# Autodesk Inventor assembly: LeftArm
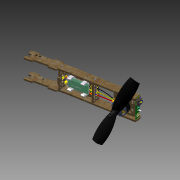
[picture p0: Inventor's stored thumbnail of the model, 180x180]
Saved by Autodesk Inventor 2012 (Build 160160000, 160)
## iProperties
Created: 2014-07-20
Part Number: LeftArm
Document SubType Name: Assembly
Designer: Anon
Author: Anon
## Documents named in this file (12)
- D:\Dropbox\Courses\GP\Inventor\dronestructure\LeftArm.iam
- D:\Dropbox\Courses\GP\Inventor\dronestructure\MotorCableHolder.ipt
- D:\Dropbox\Courses\GP\Inventor\dronestructure\ESCcableHolder.ipt
- D:\Dropbox\Courses\GP\Inventor\dronestructure\ArmOutside.ipt
- D:\Dropbox\Courses\GP\Inventor\dronestructure\ArmInsideLow.ipt
- C:\Users\Anon\Documents\Inventor\Content Center Files\R2012\en-US\ISO 4032(2)\ISO 4032 - M2,5ISO.ipt
- C:\Users\Anon\Documents\Inventor\Content Center Files\R2012\en-US\ISO 1207(1)\ISO 1207 - M2,5 x 14DIN EN ISO.ipt
- D:\Dropbox\Courses\GP\Inventor\dronestructure\electronics\afroesc\escassembly.iam
- D:\Dropbox\Courses\GP\Inventor\dronestructure\motor\motormounted.iam
- D:\Dropbox\Courses\GP\Inventor\dronestructure\LeftArm\AIP\Cable and Harness\LeftArm.MotorCables.iam
- D:\Dropbox\Courses\GP\Inventor\dronestructure\electronics\wingleds\wingledpcb\WingLeds.iam
- D:\Dropbox\Courses\GP\Inventor\dronestructure\CrimpSocket.ipt
## Components (21 placed, 11 different names)
1. MotorCableHolder:1 — Mate:19, Mate:21, Mate:27, Flush:3, Mate:28
2. ESCcableHolder:1 — Flush:1, Mate:1, Mate:2, Mate:4, Mate:5, Flush:2, Mate:11, Mate:23, Flush:5, Flush:6, Flush:7
3. ArmOutside:1 — Flush:1, Mate:1, Mate:2, Mate:8, Mate:9, Mate:12, Mate:13, Mate:25, Mate:26, Flush:3, Mate:28, Mate:31, Mate:34, Mate:35, Mate:41, Flush:4
4. ArmInsideLow:1 — Mate:4, Mate:5, Flush:2, Mate:14, Mate:15, Mate:16, Mate:17, Mate:24, Mate:27, Mate:29, Mate:30, Mate:32, Mate:33, Mate:40
5. ISO 4032 M2,5:1 — Mate:10, Mate:11
6. ISO 4032 M2,5:2 — Mate:18, Mate:19
7. ISO 4032 M2,5:3 — Mate:22, Mate:23
8. ISO 4032 M2,5:4 — Mate:20, Mate:21
9. DIN EN ISO 1207 M2,5 x 14:1 — Mate:8, Mate:9, Mate:10
10. DIN EN ISO 1207 M2,5 x 14:2 — Mate:12, Mate:13, Mate:18
11. DIN EN ISO 1207 M2,5 x 14:3 — Mate:14, Mate:15, Mate:22
12. DIN EN ISO 1207 M2,5 x 14:4 — Mate:16, Mate:17, Mate:20
13. ESC [sub-assembly] — Mate:24, Mate:25, Mate:26
14. Motor [sub-assembly] — Mate:29, Mate:30, Mate:31, Mate:37, Mate:39
15. LeftArm.MotorCables [sub-assembly]
16. DIN EN ISO 1207 M2,5 x 14:5 — Mate:32, Mate:33, Mate:38
17. DIN EN ISO 1207 M2,5 x 14:6 — Mate:34, Mate:35, Mate:36
18. ISO 4032 M2,5:5 — Mate:36, Mate:37
19. ISO 4032 M2,5:6 — Mate:38, Mate:39
20. WingLEDs [sub-assembly] — Mate:40, Mate:41, Flush:4
21. CrimpSocket:1 — Flush:5, Flush:6, Flush:7
## Relationships (45: Mate 38, Flush 7)
- Flush:1: ESCcableHolder:1 ↔ ArmOutside:1
- Mate:1: ESCcableHolder:1 ↔ ArmOutside:1
- Mate:2: ESCcableHolder:1 ↔ ArmOutside:1
- Mate:4: ESCcableHolder:1 ↔ ArmInsideLow:1
- Mate:5: ESCcableHolder:1 ↔ ArmInsideLow:1
- Flush:2: ESCcableHolder:1 ↔ ArmInsideLow:1
- Mate:8: ArmOutside:1 ↔ DIN EN ISO 1207 M2,5 x 14:1
- Mate:9: ArmOutside:1 ↔ DIN EN ISO 1207 M2,5 x 14:1
- Mate:10: ISO 4032 M2,5:1 ↔ DIN EN ISO 1207 M2,5 x 14:1
- Mate:11: ESCcableHolder:1 ↔ ISO 4032 M2,5:1
- Mate:12: ArmOutside:1 ↔ DIN EN ISO 1207 M2,5 x 14:2
- Mate:13: ArmOutside:1 ↔ DIN EN ISO 1207 M2,5 x 14:2
- Mate:14: ArmInsideLow:1 ↔ DIN EN ISO 1207 M2,5 x 14:3
- Mate:15: ArmInsideLow:1 ↔ DIN EN ISO 1207 M2,5 x 14:3
- Mate:16: ArmInsideLow:1 ↔ DIN EN ISO 1207 M2,5 x 14:4
- Mate:17: ArmInsideLow:1 ↔ DIN EN ISO 1207 M2,5 x 14:4
- Mate:18: ISO 4032 M2,5:2 ↔ DIN EN ISO 1207 M2,5 x 14:2
- Mate:19: MotorCableHolder:1 ↔ ISO 4032 M2,5:2
- Mate:20: ISO 4032 M2,5:4 ↔ DIN EN ISO 1207 M2,5 x 14:4
- Mate:21: MotorCableHolder:1 ↔ ISO 4032 M2,5:4
- Mate:22: ISO 4032 M2,5:3 ↔ DIN EN ISO 1207 M2,5 x 14:3
- Mate:23: ESCcableHolder:1 ↔ ISO 4032 M2,5:3
- Mate:24: ArmInsideLow:1 ↔ ESC
- Mate:25: ArmOutside:1 ↔ ESC
- Mate:26: ArmOutside:1 ↔ ESC
- Mate:27: MotorCableHolder:1 ↔ ArmInsideLow:1
- Flush:3: MotorCableHolder:1 ↔ ArmOutside:1
- Mate:28: MotorCableHolder:1 ↔ ArmOutside:1
- Mate:29: ArmInsideLow:1 ↔ Motor
- Mate:30: ArmInsideLow:1 ↔ Motor
- Mate:31: ArmOutside:1 ↔ Motor
- Mate:32: ArmInsideLow:1 ↔ DIN EN ISO 1207 M2,5 x 14:5
- Mate:33: ArmInsideLow:1 ↔ DIN EN ISO 1207 M2,5 x 14:5
- Mate:34: ArmOutside:1 ↔ DIN EN ISO 1207 M2,5 x 14:6
- Mate:35: ArmOutside:1 ↔ DIN EN ISO 1207 M2,5 x 14:6
- Mate:36: DIN EN ISO 1207 M2,5 x 14:6 ↔ ISO 4032 M2,5:5
- Mate:37: Motor ↔ ISO 4032 M2,5:5
- Mate:38: DIN EN ISO 1207 M2,5 x 14:5 ↔ ISO 4032 M2,5:6
- Mate:39: Motor ↔ ISO 4032 M2,5:6
- Mate:40: ArmInsideLow:1 ↔ WingLEDs
- Mate:41: ArmOutside:1 ↔ WingLEDs
- Flush:4: ArmOutside:1 ↔ WingLEDs
- Flush:5: ESCcableHolder:1 ↔ CrimpSocket:1
- Flush:6: ESCcableHolder:1 ↔ CrimpSocket:1
- Flush:7: ESCcableHolder:1 ↔ CrimpSocket:1
